# Autodesk Inventor assembly: UBG-Schutz
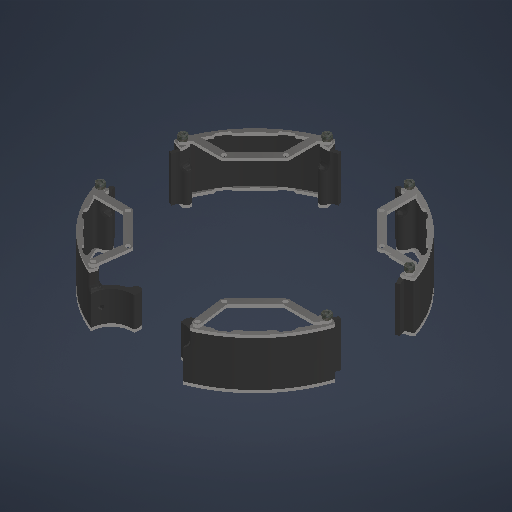
[picture p0: Inventor's stored thumbnail of the model, 512x512]
Saved by Autodesk Inventor 2025.2 (Build 292293000, 293)
## iProperties
Created: 2025-03-27
Part Number: UBG-Schutz
Document SubType Name: Assembly
Designer: Faabs
Author: Faabs
## Documents named in this file (9)
- C:\Users\Faabs\Desktop\TeamFaabs-CAD v2023\UBG\Schutz\UBG-Schutz.iam
- C:\Users\Faabs\Desktop\TeamFaabs-CAD v2023\UBG\Schutz\Schutzkoerper.ipt
- C:\Users\Faabs\Desktop\TeamFaabs-CAD v2023\UBG\Schutz\Schutzring_oben.ipt
- C:\Users\Faabs\Desktop\TeamFaabs-CAD v2023\Verbindungselemente\Inventor\M3 Schmelzgewinde\M3 Schmelzgewinde\M3 Schmelzgewinde.ipt
- C:\Users\Faabs\Desktop\TeamFaabs-CAD v2023\UBG\Schutz\Schutzring_unten.ipt
- C:\Users\Faabs\Desktop\TeamFaabs-CAD v2023\UBG\Schutz\Stabilisator_vorne.ipt
- C:\Users\Faabs\Desktop\TeamFaabs-CAD v2023\UBG\Schutz\Stabilisator_hinten.ipt
- C:\Users\Faabs\Desktop\TeamFaabs-CAD v2023\UBG\Schutz\Stabilisator_Teensy.ipt
- C:\Users\Faabs\Desktop\TeamFaabs-CAD v2023\Verbindungselemente\Inventor\DIN 912\DIN 912 - M3 x 0,5 x 8 x 6,75.ipt
## Components (29 placed, 8 different names)
1. Schutzkoerper:1 — Passend:1, Passend:2, Passend:3, Passend:4, Passend:5, Passend:6, Passend:7, Passend:8, Passend:9, Passend:10, Passend:11, Passend:12, Passend:13, Passend:14, Passend:15, Passend:16, Passend:17, Passend:18, Passend:19, Fluchtend:1, Fluchtend:2, Fluchtend:3, Fluchtend:4, Fluchtend:5, Fluchtend:6, Fluchtend:7, Fluchtend:8, Fluchtend:9, Fluchtend:10, Fluchtend:11, Fluchtend:12, Fluchtend:13, Fluchtend:14, Fluchtend:15, Fluchtend:16, Passend:22, Passend:25
2. Schutzring_oben:1 — Passend:20, Passend:21, Passend:22, Passend:26, Passend:27, Passend:28, Passend:29, Passend:30, Passend:31, Passend:32, Passend:33, Passend:34, Passend:35, Passend:36, Passend:37
3. Schutzring_unten:1 — Passend:23, Passend:24, Passend:25
4. Stabilisator_vorne:1 — Passend:26, Passend:27, Passend:28, Einfügen:2
5. Stabilisator_vorne:2 — Passend:29, Passend:30, Passend:31, Einfügen:1
6. Stabilisator_hinten:1 — Passend:34, Passend:35, Passend:36, Einfügen:5, Einfügen:6
7. Stabilisator_Teensy:1 — Passend:32, Passend:33, Passend:37, Einfügen:3, Einfügen:4
8. M3 Schmelzgewinde:1 — Passend:4, Fluchtend:16, Passend:20
9. M3 Schmelzgewinde:2 — Passend:5, Fluchtend:14
10. M3 Schmelzgewinde:3 — Passend:6, Fluchtend:15
11. M3 Schmelzgewinde:4 — Passend:7, Fluchtend:13
12. M3 Schmelzgewinde:5 — Passend:8, Fluchtend:12, Passend:21
13. M3 Schmelzgewinde:6 — Passend:9, Fluchtend:11
14. M3 Schmelzgewinde:7 — Passend:10, Fluchtend:10
15. M3 Schmelzgewinde:8 — Passend:11, Fluchtend:9
16. M3 Schmelzgewinde:9 — Passend:19, Fluchtend:1
17. M3 Schmelzgewinde:10 — Passend:18, Fluchtend:2
18. M3 Schmelzgewinde:11 — Passend:13, Fluchtend:7
19. M3 Schmelzgewinde:12 — Passend:15, Fluchtend:5, Passend:24
20. M3 Schmelzgewinde:13 — Passend:17, Fluchtend:3
21. M3 Schmelzgewinde:14 — Passend:16, Fluchtend:4
22. M3 Schmelzgewinde:15 — Passend:14, Fluchtend:6
23. M3 Schmelzgewinde:16 — Passend:12, Fluchtend:8, Passend:23
24. DIN 912 - ersetzt durch DIN EN ISO 4762 M3 x 8:1 — Einfügen:1
25. DIN 912 - ersetzt durch DIN EN ISO 4762 M3 x 8:2 — Einfügen:2
26. DIN 912 - ersetzt durch DIN EN ISO 4762 M3 x 8:3 — Einfügen:6
27. DIN 912 - ersetzt durch DIN EN ISO 4762 M3 x 8:4 — Einfügen:5
28. DIN 912 - ersetzt durch DIN EN ISO 4762 M3 x 8:6 — Einfügen:4
29. DIN 912 - ersetzt durch DIN EN ISO 4762 M3 x 8:7 — Einfügen:3
## Relationships (59: Mate 37, Flush 16, Insert 6)
- Passend:1 [Mate]: Schutzkoerper:1
- Passend:2 [Mate]: Schutzkoerper:1
- Passend:3 [Mate]: Schutzkoerper:1
- Passend:4 [Mate]: Schutzkoerper:1 ↔ M3 Schmelzgewinde:1
- Passend:5 [Mate]: Schutzkoerper:1 ↔ M3 Schmelzgewinde:2
- Passend:6 [Mate]: Schutzkoerper:1 ↔ M3 Schmelzgewinde:3
- Passend:7 [Mate]: Schutzkoerper:1 ↔ M3 Schmelzgewinde:4
- Passend:8 [Mate]: Schutzkoerper:1 ↔ M3 Schmelzgewinde:5
- Passend:9 [Mate]: Schutzkoerper:1 ↔ M3 Schmelzgewinde:6
- Passend:10 [Mate]: Schutzkoerper:1 ↔ M3 Schmelzgewinde:7
- Passend:11 [Mate]: Schutzkoerper:1 ↔ M3 Schmelzgewinde:8
- Passend:12 [Mate]: Schutzkoerper:1 ↔ M3 Schmelzgewinde:16
- Passend:13 [Mate]: Schutzkoerper:1 ↔ M3 Schmelzgewinde:11
- Passend:14 [Mate]: Schutzkoerper:1 ↔ M3 Schmelzgewinde:15
- Passend:15 [Mate]: Schutzkoerper:1 ↔ M3 Schmelzgewinde:12
- Passend:16 [Mate]: Schutzkoerper:1 ↔ M3 Schmelzgewinde:14
- Passend:17 [Mate]: Schutzkoerper:1 ↔ M3 Schmelzgewinde:13
- Passend:18 [Mate]: Schutzkoerper:1 ↔ M3 Schmelzgewinde:10
- Passend:19 [Mate]: Schutzkoerper:1 ↔ M3 Schmelzgewinde:9
- Fluchtend:1 [Flush] (0.1 mm): Schutzkoerper:1 ↔ M3 Schmelzgewinde:9
- Fluchtend:2 [Flush] (0.1 mm): Schutzkoerper:1 ↔ M3 Schmelzgewinde:10
- Fluchtend:3 [Flush] (0.1 mm): Schutzkoerper:1 ↔ M3 Schmelzgewinde:13
- Fluchtend:4 [Flush] (0.1 mm): Schutzkoerper:1 ↔ M3 Schmelzgewinde:14
- Fluchtend:5 [Flush] (0.1 mm): Schutzkoerper:1 ↔ M3 Schmelzgewinde:12
- Fluchtend:6 [Flush] (0.1 mm): Schutzkoerper:1 ↔ M3 Schmelzgewinde:15
- Fluchtend:7 [Flush] (0.1 mm): Schutzkoerper:1 ↔ M3 Schmelzgewinde:11
- Fluchtend:8 [Flush] (0.1 mm): Schutzkoerper:1 ↔ M3 Schmelzgewinde:16
- Fluchtend:9 [Flush] (0.1 mm): Schutzkoerper:1 ↔ M3 Schmelzgewinde:8
- Fluchtend:10 [Flush] (0.1 mm): Schutzkoerper:1 ↔ M3 Schmelzgewinde:7
- Fluchtend:11 [Flush] (0.1 mm): Schutzkoerper:1 ↔ M3 Schmelzgewinde:6
- Fluchtend:12 [Flush] (0.1 mm): Schutzkoerper:1 ↔ M3 Schmelzgewinde:5
- Fluchtend:13 [Flush] (0.1 mm): Schutzkoerper:1 ↔ M3 Schmelzgewinde:4
- Fluchtend:14 [Flush] (0.1 mm): Schutzkoerper:1 ↔ M3 Schmelzgewinde:2
- Fluchtend:15 [Flush] (0.1 mm): Schutzkoerper:1 ↔ M3 Schmelzgewinde:3
- Fluchtend:16 [Flush] (0.1 mm): Schutzkoerper:1 ↔ M3 Schmelzgewinde:1
- Passend:20 [Mate]: Schutzring_oben:1 ↔ M3 Schmelzgewinde:1
- Passend:21 [Mate]: Schutzring_oben:1 ↔ M3 Schmelzgewinde:5
- Passend:22 [Mate]: Schutzkoerper:1 ↔ Schutzring_oben:1
- Passend:23 [Mate]: Schutzring_unten:1 ↔ M3 Schmelzgewinde:16
- Passend:24 [Mate]: Schutzring_unten:1 ↔ M3 Schmelzgewinde:12
- Passend:25 [Mate]: Schutzkoerper:1 ↔ Schutzring_unten:1
- Passend:26 [Mate]: Schutzring_oben:1 ↔ Stabilisator_vorne:1
- Passend:27 [Mate]: Schutzring_oben:1 ↔ Stabilisator_vorne:1
- Passend:28 [Mate]: Schutzring_oben:1 ↔ Stabilisator_vorne:1
- Passend:29 [Mate]: Schutzring_oben:1 ↔ Stabilisator_vorne:2
- Passend:30 [Mate]: Schutzring_oben:1 ↔ Stabilisator_vorne:2
- Passend:31 [Mate]: Schutzring_oben:1 ↔ Stabilisator_vorne:2
- Passend:32 [Mate]: Schutzring_oben:1 ↔ Stabilisator_Teensy:1
- Passend:33 [Mate]: Schutzring_oben:1 ↔ Stabilisator_Teensy:1
- Passend:34 [Mate]: Schutzring_oben:1 ↔ Stabilisator_hinten:1
- Passend:35 [Mate]: Schutzring_oben:1 ↔ Stabilisator_hinten:1
- Passend:36 [Mate]: Schutzring_oben:1 ↔ Stabilisator_hinten:1
- Passend:37 [Mate]: Schutzring_oben:1 ↔ Stabilisator_Teensy:1
- Einfügen:1 [Insert]: Stabilisator_vorne:2 ↔ DIN 912 - ersetzt durch DIN EN ISO 4762 M3 x 8:1
- Einfügen:2 [Insert]: Stabilisator_vorne:1 ↔ DIN 912 - ersetzt durch DIN EN ISO 4762 M3 x 8:2
- Einfügen:3 [Insert]: Stabilisator_Teensy:1 ↔ DIN 912 - ersetzt durch DIN EN ISO 4762 M3 x 8:7
- Einfügen:4 [Insert]: Stabilisator_Teensy:1 ↔ DIN 912 - ersetzt durch DIN EN ISO 4762 M3 x 8:6
- Einfügen:5 [Insert]: Stabilisator_hinten:1 ↔ DIN 912 - ersetzt durch DIN EN ISO 4762 M3 x 8:4
- Einfügen:6 [Insert]: Stabilisator_hinten:1 ↔ DIN 912 - ersetzt durch DIN EN ISO 4762 M3 x 8:3
